# Autodesk Inventor assembly: neopixel_6xled_strip
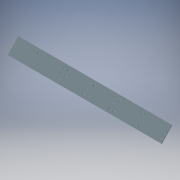
[picture p0: Inventor's stored thumbnail of the model, 180x180]
Saved by Autodesk Inventor 2016 (Build 200138000, 138)
## iProperties
Created: 2018-02-27
Part Number: neopixel_6xled_strip
Document SubType Name: Assembly
Designer: Davide
Author: Davide
## Documents named in this file (2)
- C:\Users\Davide\Documents\Inventor\Cottini Lamp\neopixel_6xled_strip.iam
- C:\Users\Davide\Documents\Inventor\Cottini Lamp\WS2812 60 per meter strip.iam
## Components (6 placed, 1 different names)
1. WS2812 60 per meter strip:1 [sub-assembly] — Mate:9, Mate:10
2. WS2812 60 per meter strip:2 [sub-assembly] — Mate:7, Mate:8, Mate:9, Mate:10
3. WS2812 60 per meter strip:3 [sub-assembly] — Mate:5, Mate:6, Mate:7, Mate:8
4. WS2812 60 per meter strip:4 [sub-assembly] — Mate:3, Mate:4, Mate:5, Mate:6
5. WS2812 60 per meter strip:5 [sub-assembly] — Mate:1, Mate:2, Mate:3, Mate:4
6. WS2812 60 per meter strip:6 [sub-assembly] — Mate:1, Mate:2
## Relationships (10: Mate 10)
- Mate:1: WS2812 60 per meter strip:5 ↔ WS2812 60 per meter strip:6
- Mate:2: WS2812 60 per meter strip:5 ↔ WS2812 60 per meter strip:6
- Mate:3: WS2812 60 per meter strip:4 ↔ WS2812 60 per meter strip:5
- Mate:4: WS2812 60 per meter strip:4 ↔ WS2812 60 per meter strip:5
- Mate:5: WS2812 60 per meter strip:3 ↔ WS2812 60 per meter strip:4
- Mate:6: WS2812 60 per meter strip:3 ↔ WS2812 60 per meter strip:4
- Mate:7: WS2812 60 per meter strip:2 ↔ WS2812 60 per meter strip:3
- Mate:8: WS2812 60 per meter strip:2 ↔ WS2812 60 per meter strip:3
- Mate:9: WS2812 60 per meter strip:1 ↔ WS2812 60 per meter strip:2
- Mate:10: WS2812 60 per meter strip:1 ↔ WS2812 60 per meter strip:2
